# Autodesk Inventor assembly: 3 Motor Gearbox
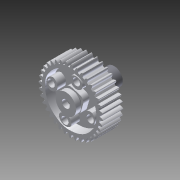
[picture p0: Inventor's stored thumbnail of the model, 180x180]
Saved by Autodesk Inventor 2014 SP1 (Build 180222100, 222)
## iProperties
Created: 2013-10-10
Part Number: 3 Motor Gearbox
Document SubType Name: Assembly
Designer: RyanHughes
Author: Andrew
Title: E:\My Documents\Inventor\VEX Robots\Sack Attack\15 defense\3 Motor Gearbox.stp
Creation Date: 2013-01-16
Sending System: Autodesk Inventor 2013
Preprocessor: Autodesk Inventor 2013
Author: RyanHughes
## Documents named in this file (5)
- C:\Users\Ryan\Desktop\sw\toss up 2ed A bot\drivetrain\gear for gearbox.iam
- C:\Users\Ryan\Desktop\sw\lib\Aperture VEX CAD Library\Gears\High Strength Gears\36 Tooth Round Insert.iam
- C:\Users\Ryan\Desktop\sw\lib\Aperture VEX CAD Library\Spacers\SPACER-0500-0125.ipt
- C:\Users\Ryan\Desktop\sw\lib\Aperture VEX CAD Library\Hardware\Shaft Collar.ipt
- C:\Users\Ryan\Desktop\sw\lib\Aperture VEX CAD Library\Spacers\SPACER-0500-0625.ipt
## Components (5 placed, 4 different names)
1. 36 Tooth Round Insert:3 [sub-assembly] — Mate:28, Mate:29, Mate:30, Mate:33
2. SPACER-0500-0125:3 — Mate:29, Mate:30, Mate:34, Mate:35
3. SPACER-0500-0125:4 — Mate:28, Mate:33
4. SPACER-0500-0625:1 — Mate:15, Mate:16, Mate:34
5. Shaft Collar:7 — Mate:15, Mate:16, Mate:35
## Relationships (8: Mate 8)
- Mate:15: SPACER-0500-0625:1 ↔ Shaft Collar:7
- Mate:16: SPACER-0500-0625:1 ↔ Shaft Collar:7
- Mate:28: 36 Tooth Round Insert:3 ↔ SPACER-0500-0125:4
- Mate:29: 36 Tooth Round Insert:3 ↔ SPACER-0500-0125:3
- Mate:30: 36 Tooth Round Insert:3 ↔ SPACER-0500-0125:3
- Mate:33: 36 Tooth Round Insert:3 ↔ SPACER-0500-0125:4
- Mate:34 (3.175 mm): SPACER-0500-0125:3 ↔ SPACER-0500-0625:1
- Mate:35: SPACER-0500-0125:3 ↔ Shaft Collar:7
